# Autodesk Inventor assembly: assemlby
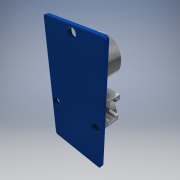
[picture p0: Inventor's stored thumbnail of the model, 180x180]
Saved by Autodesk Inventor 2019.4 (Build 234330000, 330)
## iProperties
Created: 2020-01-12
Part Number: assemlby
Material: Générique
Document SubType Name: Assembly
Designer: thoma
Author: thoma
## Documents named in this file (4)
- C:\Users\thoma\Documents\GrabCAD\smart-bowl\ultrasonic_ranger\assemlby.iam
- C:\Users\thoma\Documents\GrabCAD\smart-bowl\ultrasonic_ranger\PCB.ipt
- C:\Users\thoma\Documents\GrabCAD\smart-bowl\ultrasonic_ranger\sensor.ipt
- C:\Users\thoma\Documents\GrabCAD\smart-bowl\actuators\Grove_micro_switch_v1.0\Grove_L_connector.ipt
## Components (4 placed, 3 different names)
1. PCB:1 — Affleurement:3, Placage:2, Affleurement:4, Placage:3, Placage:5, Affleurement:5, Placage:6
2. sensor:1 — Affleurement:3, Placage:3, Placage:4, Placage:5
3. sensor:2 — Placage:2, Affleurement:4, Placage:4
4. Grove_L_connector:1 — Affleurement:5, Placage:6
## Relationships (8: Mate 5, Flush 3)
- Affleurement:3 [Flush]: PCB:1 ↔ sensor:1
- Placage:2 [Mate]: PCB:1 ↔ sensor:2
- Affleurement:4 [Flush] (12.5 mm): PCB:1 ↔ sensor:2
- Placage:3 [Mate] (-12.5 mm): PCB:1 ↔ sensor:1
- Placage:4 [Mate] (22 mm): sensor:1 ↔ sensor:2
- Placage:5 [Mate] (-14 mm): PCB:1 ↔ sensor:1
- Affleurement:5 [Flush] (-1 mm): PCB:1 ↔ Grove_L_connector:1
- Placage:6 [Mate]: PCB:1 ↔ Grove_L_connector:1
